# Autodesk Inventor assembly: z_axys_extrusorù
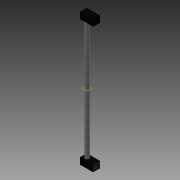
[picture p0: Inventor's stored thumbnail of the model, 180x180]
Saved by Autodesk Inventor 2014 SP1 (Build 180222100, 222)
## iProperties
Created: 2015-04-08
Part Number: z_axys_extrusorù
Document SubType Name: Assembly
Designer: Giorgio Nuzzo
Author: Giorgio Nuzzo
## Documents named in this file (4)
- C:\Users\Giorgio Nuzzo\Desktop\3dragmodel\z_axys_extrusorù.iam
- C:\Users\Giorgio Nuzzo\Desktop\3dragmodel\supporto_guide_10Z.ipt
- C:\Users\Giorgio Nuzzo\Desktop\3dragmodel\guida_Z.ipt
- C:\Users\Giorgio Nuzzo\Desktop\3dragmodel\supporto_guide_10Z_MIR.ipt
## Components (3 placed, 3 different names)
1. supporto_guide_10Z:1 — Insert:2, Flush:1
2. guida_Z:1 — Insert:1, Insert:2
3. supporto_guide_10Z_MIR:1 — Mate:2, Insert:1, Flush:1
## Relationships (4: Insert 2, Mate 1, Flush 1)
- Mate:2: supporto_guide_10Z_MIR:1
- Insert:1: guida_Z:1 ↔ supporto_guide_10Z_MIR:1
- Insert:2: supporto_guide_10Z:1 ↔ guida_Z:1
- Flush:1: supporto_guide_10Z:1 ↔ supporto_guide_10Z_MIR:1
